# Autodesk Inventor assembly: Drive
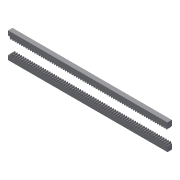
[picture p0: Inventor's stored thumbnail of the model, 180x180]
Saved by Autodesk Inventor 2016 (Build 200138000, 138)
## iProperties
Created: 2016-04-05
Part Number: Drive
Document SubType Name: Assembly
Designer: Ariana
Author: Ariana
## Documents named in this file (3)
- C:\Users\Ariana\Downloads\Capstone CAD\Capstone CAD\Delivery\Drive.iam
- C:\Users\Ariana\Downloads\Capstone CAD\Capstone CAD\Delivery\Drive Frame.ipt
- C:\Users\Ariana\Downloads\Capstone CAD\Capstone CAD\Delivery\Full Rack.iam
## Components (4 placed, 2 different names)
1. Drive Frame:1 — Flush:1, Flush:2, Flush:3, Mate:1, Flush:4, Flush:5, Flush:7, Flush:8
2. Full Rack:1 [sub-assembly] — Mate:1, Flush:4, Flush:5, Mate:2
3. Full Rack:2 [sub-assembly] — Mate:2, Flush:7, Flush:8, Mate:3, Flush:9, Flush:10
4. Drive Frame:2 — Mate:3, Flush:9, Flush:10
## Relationships (12: Flush 9, Mate 3)
- Flush:1: Drive Frame:1
- Flush:2: Drive Frame:1
- Flush:3: Drive Frame:1
- Mate:1: Drive Frame:1 ↔ Full Rack:1
- Flush:4: Drive Frame:1 ↔ Full Rack:1
- Flush:5: Drive Frame:1 ↔ Full Rack:1
- Mate:2 (35.0012 mm): Full Rack:1 ↔ Full Rack:2
- Flush:7: Drive Frame:1 ↔ Full Rack:2
- Flush:8: Drive Frame:1 ↔ Full Rack:2
- Mate:3: Full Rack:2 ↔ Drive Frame:2
- Flush:9: Full Rack:2 ↔ Drive Frame:2
- Flush:10: Full Rack:2 ↔ Drive Frame:2
